# Autodesk Inventor assembly: sub_flap
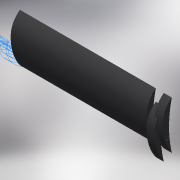
[picture p0: Inventor's stored thumbnail of the model, 180x180]
Saved by Autodesk Inventor 2018.2 (Build 222227000, 227)
## iProperties
Created: 2017-12-11
Part Number: sub_flap
Material: 一般
Document SubType Name: Assembly
Designer: kuwano
Mass: 5350.49 g
Surface Area: 6649.29 cm^2
Volume: 5240.44 cm^3
Density: 1.021 g/cm^3
Author: kuwano
## Documents named in this file (3)
- D:\kuwano\Documents\Inventor\KITformula\AeroCAD2018\CAD\Inventor\製作用CAD\R-wing\parts\sub_flap\sub_flap.iam
- D:\kuwano\Documents\Inventor\KITformula\AeroCAD2018\CAD\Inventor\製作用CAD\R-wing\parts\sub_flap\parts\styro_50_sub.ipt
- D:\kuwano\Documents\Inventor\KITformula\AeroCAD2018\CAD\Inventor\製作用CAD\R-wing\parts\sub_flap\parts\pipe.ipt
## Components (20 placed, 2 different names)
1. styro_50_sub:1 — メイト:1, メイト:2, メイト:37
2. styro_50_sub:2 — メイト:1, メイト:2, メイト:5, メイト:6, メイト:37, メイト:38
3. styro_50_sub:3 — メイト:5, メイト:6, メイト:38, メイト:39
4. styro_50_sub:4 — メイト:13, メイト:14, メイト:39, メイト:40
5. styro_50_sub:5 — メイト:13, メイト:14, メイト:40, メイト:41
6. styro_50_sub:6 — メイト:41, メイト:42
7. styro_50_sub:7 — メイト:42, メイト:43
8. styro_50_sub:8 — メイト:29, メイト:30, メイト:43, メイト:44
9. styro_50_sub:9 — メイト:29, メイト:30, メイト:44, メイト:45
10. styro_50_sub:10 — メイト:45, メイト:46, フラッシュ:1
11. styro_50_sub:11 — メイト:46, メイト:47
12. styro_50_sub:12 — メイト:47, メイト:48
13. styro_50_sub:13 — メイト:48, メイト:49
14. styro_50_sub:14 — メイト:49, メイト:50
15. styro_50_sub:15 — メイト:50, メイト:51
16. styro_50_sub:16 — メイト:35, メイト:36, メイト:51, メイト:52
17. styro_50_sub:17 — メイト:35, メイト:36, メイト:52, メイト:53
18. styro_50_sub:18 — メイト:53, メイト:54
19. styro_50_sub:19 — メイト:54, メイト:55, フラッシュ:2
20. pipe:1 — メイト:55, フラッシュ:2
## Relationships (57: Mate 55, Flush 2)
- メイト:1 [Mate]: styro_50_sub:1 ↔ styro_50_sub:2
- メイト:2 [Mate]: styro_50_sub:1 ↔ styro_50_sub:2
- [Mate]: styro_50_sub:3 ↔ styro_50_sub:4
- [Mate]: styro_50_sub:3 ↔ styro_50_sub:4
- メイト:5 [Mate]: styro_50_sub:2 ↔ styro_50_sub:3
- メイト:6 [Mate]: styro_50_sub:2 ↔ styro_50_sub:3
- [Mate]: styro_50_sub:5 ↔ styro_50_sub:6
- [Mate]: styro_50_sub:5 ↔ styro_50_sub:6
- [Mate]: styro_50_sub:7 ↔ styro_50_sub:8
- [Mate]: styro_50_sub:7 ↔ styro_50_sub:8
- [Mate]: styro_50_sub:6 ↔ styro_50_sub:7
- [Mate]: styro_50_sub:6 ↔ styro_50_sub:7
- メイト:13 [Mate]: styro_50_sub:4 ↔ styro_50_sub:5
- メイト:14 [Mate]: styro_50_sub:4 ↔ styro_50_sub:5
- [Mate]: styro_50_sub:9 ↔ styro_50_sub:10
- [Mate]: styro_50_sub:9 ↔ styro_50_sub:10
- [Mate]: styro_50_sub:11 ↔ styro_50_sub:12
- [Mate]: styro_50_sub:11 ↔ styro_50_sub:12
- [Mate]: styro_50_sub:10 ↔ styro_50_sub:11
- [Mate]: styro_50_sub:10 ↔ styro_50_sub:11
- [Mate]: styro_50_sub:13 ↔ styro_50_sub:14
- [Mate]: styro_50_sub:13 ↔ styro_50_sub:14
- [Mate]: styro_50_sub:15 ↔ styro_50_sub:16
- [Mate]: styro_50_sub:15 ↔ styro_50_sub:16
- [Mate]: styro_50_sub:14 ↔ styro_50_sub:15
- [Mate]: styro_50_sub:14 ↔ styro_50_sub:15
- [Mate]: styro_50_sub:12 ↔ styro_50_sub:13
- [Mate]: styro_50_sub:12 ↔ styro_50_sub:13
- メイト:29 [Mate]: styro_50_sub:8 ↔ styro_50_sub:9
- メイト:30 [Mate]: styro_50_sub:8 ↔ styro_50_sub:9
- [Mate]: styro_50_sub:18 ↔ styro_50_sub:19
- [Mate]: styro_50_sub:18 ↔ styro_50_sub:19
- [Mate]: styro_50_sub:17 ↔ styro_50_sub:18
- [Mate]: styro_50_sub:17 ↔ styro_50_sub:18
- メイト:35 [Mate]: styro_50_sub:16 ↔ styro_50_sub:17
- メイト:36 [Mate]: styro_50_sub:16 ↔ styro_50_sub:17
- メイト:37 [Mate]: styro_50_sub:1 ↔ styro_50_sub:2
- メイト:38 [Mate]: styro_50_sub:2 ↔ styro_50_sub:3
- メイト:39 [Mate]: styro_50_sub:3 ↔ styro_50_sub:4
- メイト:40 [Mate]: styro_50_sub:4 ↔ styro_50_sub:5
- メイト:41 [Mate]: styro_50_sub:5 ↔ styro_50_sub:6
- メイト:42 [Mate]: styro_50_sub:6 ↔ styro_50_sub:7
- メイト:43 [Mate]: styro_50_sub:7 ↔ styro_50_sub:8
- メイト:44 [Mate]: styro_50_sub:8 ↔ styro_50_sub:9
- メイト:45 [Mate]: styro_50_sub:9 ↔ styro_50_sub:10
- メイト:46 [Mate]: styro_50_sub:10 ↔ styro_50_sub:11
- メイト:47 [Mate]: styro_50_sub:11 ↔ styro_50_sub:12
- メイト:48 [Mate]: styro_50_sub:12 ↔ styro_50_sub:13
- メイト:49 [Mate]: styro_50_sub:13 ↔ styro_50_sub:14
- メイト:50 [Mate]: styro_50_sub:14 ↔ styro_50_sub:15
- メイト:51 [Mate]: styro_50_sub:15 ↔ styro_50_sub:16
- メイト:52 [Mate]: styro_50_sub:16 ↔ styro_50_sub:17
- メイト:53 [Mate]: styro_50_sub:17 ↔ styro_50_sub:18
- メイト:54 [Mate]: styro_50_sub:18 ↔ styro_50_sub:19
- フラッシュ:1 [Flush]: styro_50_sub:10
- メイト:55 [Mate]: styro_50_sub:19 ↔ pipe:1
- フラッシュ:2 [Flush]: styro_50_sub:19 ↔ pipe:1
## Named parameters: d59_d57 = 0 mm, d60_d58 = 0 mm, d63_d57 = 0 mm, d64_d58 = 0 mm, d65_d59_d57 = 0 mm, d66_d60_d58 = 0 mm, d67_d61 = 0 mm, d68_d62 = 0 mm, d71_d69 = 0 mm, d72_d70 = 0 mm, d73_d57 = 0 mm, d74_d58 = 0 mm, d75_d59_d57 = 0 mm, d76_d60_d58 = 0 mm, d77_d61 = 0 mm, d78_d62 = 0 mm, d79_d63_d57 = 0 mm, d80_d64_d58 = 0 mm, d81_d65_d59_d57 = 0 mm, d82_d66_d60_d58 = 0 mm, d83_d67_d61 = 0 mm, d84_d68_d62 = 0 mm, d87_d81_d65_d59_d57 = 0 mm, d88_d82_d66_d60_d58 = 0 mm, d89_d83_d67_d61 = 0 mm, d90_d84_d68_d62 = 0 mm
